# Autodesk Inventor assembly: ASY Луч 1
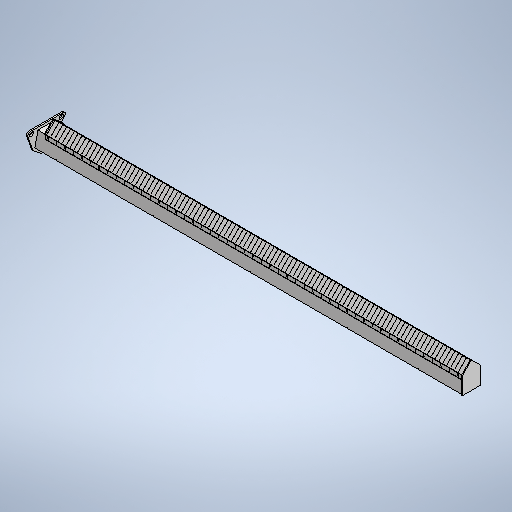
[picture p0: Inventor's stored thumbnail of the model, 512x512]
Saved by Autodesk Inventor 2025 (Build 290162010, 162A)
## iProperties
Created: 2025-02-18
Part Number: ASY Луч 1
Document SubType Name: Assembly
Designer: admin
Author: admin
## Documents named in this file (6)
- C:\Users\admin\YandexDisk-badmisterfox\home pc\Inventor\Manturovo\Manturovo_Se-clar\Дренаж на угольные\ASY Луч 1.iam
- C:\Users\admin\YandexDisk-badmisterfox\home pc\Inventor\Manturovo\Manturovo_Se-clar\Дренаж на угольные\MNT-CDF-301 beam 1.ipt
- C:\Users\admin\YandexDisk-badmisterfox\home pc\Inventor\Manturovo\Manturovo_Se-clar\Дренаж на угольные\MNT-CDF-401 roof 1.ipt
- C:\Users\admin\YandexDisk-badmisterfox\home pc\Inventor\Manturovo\Manturovo_Se-clar\Дренаж на угольные\MNT-CDF-504 small tube flange.ipt
- C:\Users\admin\YandexDisk-badmisterfox\home pc\Inventor\Manturovo\Manturovo_Se-clar\Дренаж на угольные\MNT-CDF-604 CAP.ipt
- C:\Users\admin\YandexDisk-badmisterfox\home pc\Inventor\Manturovo\Manturovo_Se-clar\Дренаж на угольные\MNT-CDF-605 CAP.ipt
## Components (5 placed, 5 different names)
1. MNT-CDF-301 beam 1:1 — Mate:2, Flush:3, Flush:4
2. MNT-CDF-401 roof 1:1
3. Part1:1
4. MNT-CDF-604 CAP:1
5. MNT-CDF-605 CAP:1
## Relationships (9: Flush 4, WeldJoint 3, Mate 2)
- [Flush]: MNT-CDF-301 beam 1:1 ↔ MNT-CDF-401 roof 1:1
- [Mate]: MNT-CDF-301 beam 1:1 ↔ MNT-CDF-401 roof 1:1
- [Flush]: MNT-CDF-301 beam 1:1 ↔ MNT-CDF-401 roof 1:1
- [WeldJoint]: MNT-CDF-301 beam 1:1 ↔ Part1:1
- [WeldJoint]: MNT-CDF-401 roof 1:1 ↔ MNT-CDF-604 CAP:1
- [WeldJoint]: MNT-CDF-401 roof 1:1 ↔ MNT-CDF-605 CAP:1
- Mate:2: MNT-CDF-301 beam 1:1
- Flush:3: MNT-CDF-301 beam 1:1
- Flush:4: MNT-CDF-301 beam 1:1
